# Autodesk Inventor assembly: 01.02.03.00 - Braço esquerdo
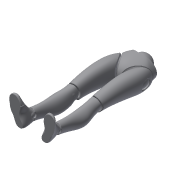
[picture p0: Inventor's stored thumbnail of the model, 180x180]
Saved by Autodesk Inventor 2016 (Build 200138000, 138)
## iProperties
Created: 2017-03-23
Part Number: 01.02.03.00 - Braço esquerdo
Document SubType Name: Assembly
Designer: Wesley Perez
Author: Wesley Perez
## Documents named in this file (4)
- D:\EMPRESARIAL\ADEBOTT\Dep. PROJETOS\ADEBOTT - KIT PROJETISTA\Corpos Humanos\Corpo Humano 01\Parts\01.01.01.00 - Membros inferiores.iam
- D:\EMPRESARIAL\ADEBOTT\Dep. PROJETOS\ADEBOTT - KIT PROJETISTA\Corpos Humanos\Corpo Humano 01\Parts\01.01.01.01 - Quadril.ipt
- D:\EMPRESARIAL\ADEBOTT\Dep. PROJETOS\ADEBOTT - KIT PROJETISTA\Corpos Humanos\Corpo Humano 01\Parts\01.01.02.00 - Perna direita.iam
- D:\EMPRESARIAL\ADEBOTT\Dep. PROJETOS\ADEBOTT - KIT PROJETISTA\Corpos Humanos\Corpo Humano 01\Parts\01.01.03.00 - Perna esquerda.iam
## Components (3 placed, 3 different names)
1. 01.01.01.01 - Quadril:1 — Alinhamento:1, Alinhamento:2, Alinhamento:3, Coincidência:1, Coincidência:2
2. 01.01.02.00 - Perna direita:1 [sub-assembly] — Coincidência:1
3. 01.01.03.00 - Perna esquerda:1 [sub-assembly] — Coincidência:2
## Relationships (5: Flush 3, Mate 2)
- Alinhamento:1 [Flush]: 01.01.01.01 - Quadril:1
- Alinhamento:2 [Flush]: 01.01.01.01 - Quadril:1
- Alinhamento:3 [Flush]: 01.01.01.01 - Quadril:1
- Coincidência:1 [Mate]: 01.01.01.01 - Quadril:1 ↔ 01.01.02.00 - Perna direita:1
- Coincidência:2 [Mate]: 01.01.01.01 - Quadril:1 ↔ 01.01.03.00 - Perna esquerda:1
